# Autodesk Inventor assembly: sensor_board
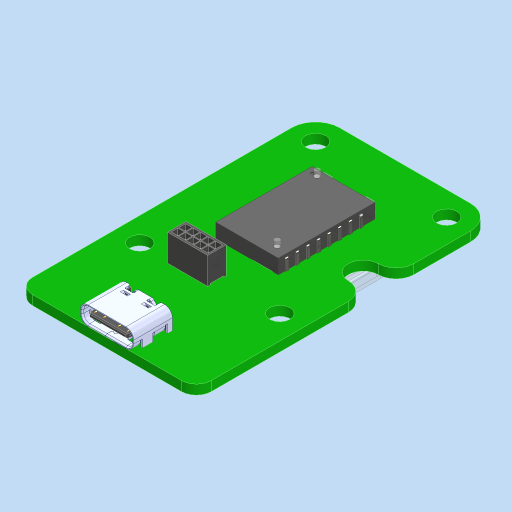
[picture p0: Inventor's stored thumbnail of the model, 512x512]
Saved by Autodesk Inventor 2024 (Build 280153000, 153)
## iProperties
Created: 2025-05-06
Part Number: sensor_board
Document SubType Name: Assembly
Designer: XxPan
Author: XxPan
## iProperties of the stored document LPPB052CFFN-RC.ipt
Created: 2022-01-18
Part Number: LPPB052CFFN-RC
Material: Generic
Description: STEP AP214
Document SubType Name: Modeling
Designer: XxPan
Density: 1 g/cm^3
Appearance: Default
Sending System: SolidWorks 2020
Preprocessor: SwSTEP 2.0
Title: LPPB052CFFN-RC.STEP
Revision Number: ANY
## iProperties of the stored document 2171790001_2171790001.ipt
Created: 2025-05-10
Part Number: 2171790001_2171790001
Material: Generic
Document SubType Name: Modeling
Designer: XxPan
Density: 1 g/cm^3
Appearance: Default
Author: XxPan
Revision Number: ANY
## iProperties of the stored document 2171790001.iam
Created: 2023-11-14
Part Number: 2171790001
Description: STEP AP214
Document SubType Name: Assembly
Designer: XxPan
Sending System: SolidWorks 2021
Preprocessor: SwSTEP 2.0
Title: 2171790001.STEP
Revision Number: ANY
## Documents named in this file (11)
- D:\The Mind Palace\remmy_mouse\CAD\sensor_board.iam
- D:\The Mind Palace\remmy_mouse\CAD\PMW3360_sensor.ipt
- D:\The Mind Palace\remmy_mouse\CAD\sensor_pcb.ipt
- D:\The Mind Palace\remmy_mouse\CAD\LM19-LSI_lens.ipt
- **D:\The Mind Palace\remmy_mouse\CAD\sensor_board.iam*LocalDocs*xAaaaqtcaAaaaaaaaAaaaadrs4g*2171790001.iam
- **D:\The Mind Palace\remmy_mouse\CAD\sensor_board.iam*LocalDocs*xAaaaqfcaAaaaaaaaAaaaq4rtNa*LPPB052CFFN-RC.ipt
- **C:\Users\XxPan\OneDrive - McMaster University\Mouse\CAD\sensor_board.iam*LocalDocs*xAaaaqfcaAaaaaaaaAaaaq4rtNa*LPPB052CFFN-RC.ipt
- **C:\Users\XxPan\OneDrive - McMaster University\Mouse\CAD\sensor_board.iam*LocalDocs*xAaaaq3caAaaaaaaaAaaaahd5Jf*2171790001_2171790001.ipt
- **C:\Users\XxPan\OneDrive - McMaster University\Mouse\CAD\sensor_board.iam*LocalDocs*xAaaaqtcaAaaaaaaaAaaaadrs4g*2171790001.iam
- D:\The Mind Palace\remmy_mouse\CAD_models\2171790001 (USB-C, 16+8 dummy, SMD, board guide)\2171790001.step
- D:\The Mind Palace\remmy_mouse\CAD_models\LPPB052CFFN_RC (2x5_P1.27mm_female_header)\LPPB052CFFN-RC.STEP
## Components (5 placed, 5 different names)
1. PMW3360_sensor:1 — Mate:1, Flush:6, Mate:24, Cylindrical:1, Angle:1, Mate:25, Mate:26
2. sensor_pcb:1 — Mate:1, Mate:21, Flush:1, Flush:2, Flush:3, Flush:4, Flush:5, Mate:22, Mate:25, Flush:7
3. LM19-LSI_lens:1 — Mate:24, Cylindrical:1, Angle:1
4. 2171790001:1 [sub-assembly] — Mate:21, Flush:2, Flush:5
5. LPPB052CFFN-RC:1 — Mate:22, Mate:26, Flush:7
## Relationships (15: Flush 7, Mate 6, CylindricalJoint 1, Angle 1)
- Mate:1: PMW3360_sensor:1 ↔ sensor_pcb:1
- Mate:21: sensor_pcb:1 ↔ 2171790001:1
- Flush:1: sensor_pcb:1
- Flush:2: sensor_pcb:1 ↔ 2171790001:1
- Flush:3: sensor_pcb:1
- Flush:4: sensor_pcb:1
- Flush:5: sensor_pcb:1 ↔ 2171790001:1
- Mate:22: sensor_pcb:1 ↔ LPPB052CFFN-RC:1
- Flush:6: PMW3360_sensor:1
- Mate:24 (-7.4 mm): PMW3360_sensor:1 ↔ LM19-LSI_lens:1
- Cylindrical:1: PMW3360_sensor:1 ↔ LM19-LSI_lens:1
- Angle:1 (0 deg): PMW3360_sensor:1 ↔ LM19-LSI_lens:1
- Mate:25: PMW3360_sensor:1 ↔ sensor_pcb:1
- Mate:26 (4.5 mm): PMW3360_sensor:1 ↔ LPPB052CFFN-RC:1
- Flush:7 (14 mm): sensor_pcb:1 ↔ LPPB052CFFN-RC:1
